# Autodesk Inventor assembly: 1103 Lift - Middle Tier
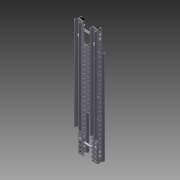
[picture p0: Inventor's stored thumbnail of the model, 180x180]
Saved by Autodesk Inventor 2012 (Build 160160000, 160)
## iProperties
Created: 2011-08-16
Part Number: 1103 Lift - Middle Tier
Document SubType Name: Assembly
Designer: Dakota.Bayer
Author: Dakota.Bayer
## Documents named in this file (11)
- C:\Users\Wade\Documents\1103 Robot - CAD Assembly\1103 Lift - Middle Tier.iam
- C:\Users\Wade\Documents\1103 Robot - CAD Assembly\Outside.ipt
- C:\Users\Wade\Documents\1103 Robot - CAD Assembly\1103 custom 5 x 30.ipt
- C:\Users\Wade\Documents\1103 Robot - CAD Assembly\Flat Bearing Block.ipt
- C:\Users\Wade\Documents\24C VEX CAD Files\Metal Other\Linear Slide Assembly-Parts\Linear Slide-Inner.ipt
- C:\Users\Wade\Documents\24C VEX CAD Files\Screws & Nuts\Screw 8-32 x 0.250''-Silver.ipt
- C:\Users\Wade\Documents\24C VEX CAD Files\Standoffs & Couplers\Standoff 0.50''.ipt
- C:\Users\Wade\Documents\1103 Robot - CAD Assembly\.5'' Screw & Nylock Nut.iam
- C:\Users\Wade\Documents\1103 Robot - CAD Assembly\.375'' Screw & Nylock Nut.iam
- C:\Users\Wade\Documents\24C VEX CAD Files\Screws & Nuts\Screw 8-32 x 0.500''-Silver.ipt
- C:\Users\Wade\Documents\24C VEX CAD Files\Standoffs & Couplers\Standoff 2.00''.ipt
## Components (35 placed, 10 different names)
1. Outside:1 — Mate:26, Flush:12, Mate:149, Mate:151
2. Outside:2 — Flush:25, Mate:153, Mate:154
3. Screw 8-32 x 0.250''-Silver:2
4. 1103 custom 5 x 30:1 — Mate:26, Flush:12, Mate:59, Mate:64, Mate:81, Mate:86, Flush:25, Mate:114, Mate:115, Mate:116, Mate:117, Mate:118, Mate:119, Mate:120, Mate:125, Mate:127, Mate:129, Mate:130, Mate:131, Mate:134, Mate:136, Mate:137, Mate:138, Mate:141, Mate:143, Mate:144, Mate:145, Mate:146, Mate:147, Mate:148, Mate:150, Mate:152, Mate:156, Mate:158, Mate:160, Mate:162
5. Standoff 0.50'':1
6. Standoff 0.50'':2
7. Standoff 0.50'':3
8. Standoff 0.50'':4
9. Linear Slide-Inner:1
10. Screw 8-32 x 0.250''-Silver:5
11. Screw 8-32 x 0.250''-Silver:6
12. Linear Slide-Inner:2
13. Screw 8-32 x 0.250''-Silver:7
14. Screw 8-32 x 0.250''-Silver:8
15. Flat Bearing Block:1 — Mate:59, Mate:118, Mate:119, Mate:120, Mate:121, Mate:161
16. Flat Bearing Block:2 — Mate:64, Mate:114, Mate:115, Mate:116, Mate:117, Mate:123, Mate:159, Mate:164
17. Flat Bearing Block:3 — Mate:81, Mate:136, Mate:137, Mate:138, Mate:139, Mate:157
18. Flat Bearing Block:4 — Mate:86, Mate:129, Mate:130, Mate:131, Mate:132, Mate:155, Mate:166
19. Screw 8-32 x 0.250''-Silver:9
20. Screw 8-32 x 0.250''-Silver:10
21. Screw 8-32 x 0.250''-Silver:11
22. .5'' Screw & Nylock Nut:1 [sub-assembly] — Mate:121, Mate:125
23. .5'' Screw & Nylock Nut:3 [sub-assembly] — Mate:123, Mate:127
24. .5'' Screw & Nylock Nut:5 [sub-assembly] — Mate:139, Mate:141
25. .5'' Screw & Nylock Nut:6 [sub-assembly] — Mate:132, Mate:134
26. Screw 8-32 x 0.500''-Silver:1 — Mate:155, Mate:156, Mate:165
27. .375'' Screw & Nylock Nut:1 [sub-assembly] — Mate:146, Mate:147, Mate:148
28. .375'' Screw & Nylock Nut:2 [sub-assembly] — Mate:143, Mate:144, Mate:145
29. .375'' Screw & Nylock Nut:3 [sub-assembly] — Mate:149, Mate:150, Mate:151
30. .375'' Screw & Nylock Nut:4 [sub-assembly] — Mate:152, Mate:153, Mate:154
31. Screw 8-32 x 0.500''-Silver:2 — Mate:157, Mate:158
32. Screw 8-32 x 0.500''-Silver:3 — Mate:161, Mate:162
33. Screw 8-32 x 0.500''-Silver:4 — Mate:159, Mate:160, Mate:163
34. Standoff 2.00'':1 — Mate:163, Mate:164
35. Standoff 2.00'':2 — Mate:165, Mate:166
## Relationships (91: Mate 76, Tangent 12, Flush 3)
- Mate:26: Outside:1 ↔ 1103 custom 5 x 30:1
- Flush:12: Outside:1 ↔ 1103 custom 5 x 30:1
- [Tangent] (0.2286 mm): Screw 8-32 x 0.250''-Silver:2 ↔ 1103 custom 5 x 30:1
- [Mate]: 1103 custom 5 x 30:1 ↔ Standoff 0.50'':1
- [Mate]: 1103 custom 5 x 30:1 ↔ Standoff 0.50'':2
- [Mate]: 1103 custom 5 x 30:1 ↔ Standoff 0.50'':3
- [Mate]: 1103 custom 5 x 30:1 ↔ Standoff 0.50'':4
- [Mate]: Screw 8-32 x 0.250''-Silver:2 ↔ Standoff 0.50'':4
- [Mate]: Standoff 0.50'':3 ↔ Linear Slide-Inner:1
- [Mate]: Linear Slide-Inner:1 ↔ Screw 8-32 x 0.250''-Silver:5
- [Tangent] (0.2286 mm): Linear Slide-Inner:1 ↔ Screw 8-32 x 0.250''-Silver:5
- [Mate]: Standoff 0.50'':1 ↔ Linear Slide-Inner:1
- [Mate]: Linear Slide-Inner:1 ↔ Screw 8-32 x 0.250''-Silver:6
- [Tangent] (0.2286 mm): Linear Slide-Inner:1 ↔ Screw 8-32 x 0.250''-Silver:6
- [Mate]: Standoff 0.50'':1 ↔ Screw 8-32 x 0.250''-Silver:6
- [Mate]: Standoff 0.50'':4 ↔ Linear Slide-Inner:2
- [Mate]: Standoff 0.50'':2 ↔ Linear Slide-Inner:2
- [Mate]: Linear Slide-Inner:2 ↔ Screw 8-32 x 0.250''-Silver:7
- [Tangent] (0.2286 mm): Linear Slide-Inner:2 ↔ Screw 8-32 x 0.250''-Silver:7
- [Mate]: Linear Slide-Inner:2 ↔ Screw 8-32 x 0.250''-Silver:8
- [Tangent] (0.2286 mm): Linear Slide-Inner:2 ↔ Screw 8-32 x 0.250''-Silver:8
- [Mate]: Standoff 0.50'':2 ↔ Screw 8-32 x 0.250''-Silver:7
- [Mate]: Standoff 0.50'':4 ↔ Screw 8-32 x 0.250''-Silver:8
- Mate:59: 1103 custom 5 x 30:1 ↔ Flat Bearing Block:1
- Mate:64: 1103 custom 5 x 30:1 ↔ Flat Bearing Block:2
- Mate:81: 1103 custom 5 x 30:1 ↔ Flat Bearing Block:3
- Mate:86: 1103 custom 5 x 30:1 ↔ Flat Bearing Block:4
- [Mate]: Standoff 0.50'':3 ↔ Screw 8-32 x 0.250''-Silver:5
- [Tangent] (0.2286 mm): Linear Slide-Inner:1 ↔ Screw 8-32 x 0.250''-Silver:6
- [Tangent] (0.2286 mm): Linear Slide-Inner:1 ↔ Screw 8-32 x 0.250''-Silver:5
- [Flush]: 1103 custom 5 x 30:1 ↔ Linear Slide-Inner:1
- [Mate]: Outside:1 ↔ Screw 8-32 x 0.250''-Silver:9
- [Tangent] (0.2286 mm): 1103 custom 5 x 30:1 ↔ Screw 8-32 x 0.250''-Silver:9
- [Tangent] (0.2286 mm): 1103 custom 5 x 30:1 ↔ Screw 8-32 x 0.250''-Silver:9
- [Mate]: Standoff 0.50'':1 ↔ Screw 8-32 x 0.250''-Silver:9
- [Mate]: Screw 8-32 x 0.250''-Silver:2 ↔ 1103 custom 5 x 30:1
- [Tangent] (0.2286 mm): Linear Slide-Inner:2 ↔ Screw 8-32 x 0.250''-Silver:8
- [Tangent] (0.2286 mm): Screw 8-32 x 0.250''-Silver:2 ↔ 1103 custom 5 x 30:1
- [Tangent] (0.2286 mm): Linear Slide-Inner:2 ↔ Screw 8-32 x 0.250''-Silver:7
- [Mate]: Outside:2 ↔ Screw 8-32 x 0.250''-Silver:10
- [Mate]: Standoff 0.50'':2 ↔ Screw 8-32 x 0.250''-Silver:10
- [Mate]: 1103 custom 5 x 30:1 ↔ Screw 8-32 x 0.250''-Silver:11
- [Mate]: Standoff 0.50'':3 ↔ Screw 8-32 x 0.250''-Silver:11
- [Mate] (2.3114 mm): 1103 custom 5 x 30:1 ↔ Standoff 0.50'':2
- [Mate] (1.1684 mm): 1103 custom 5 x 30:1 ↔ Screw 8-32 x 0.250''-Silver:10
- Flush:25: Outside:2 ↔ 1103 custom 5 x 30:1
- Mate:114 (2.3114 mm): 1103 custom 5 x 30:1 ↔ Flat Bearing Block:2
- Mate:115 (2.3114 mm): 1103 custom 5 x 30:1 ↔ Flat Bearing Block:2
- Mate:116 (2.3114 mm): 1103 custom 5 x 30:1 ↔ Flat Bearing Block:2
- Mate:117 (2.3114 mm): 1103 custom 5 x 30:1 ↔ Flat Bearing Block:2
- Mate:118 (2.3114 mm): 1103 custom 5 x 30:1 ↔ Flat Bearing Block:1
- Mate:119 (2.3114 mm): 1103 custom 5 x 30:1 ↔ Flat Bearing Block:1
- Mate:120 (2.3114 mm): 1103 custom 5 x 30:1 ↔ Flat Bearing Block:1
- Mate:121: Flat Bearing Block:1 ↔ .5'' Screw & Nylock Nut:1
- Mate:123: Flat Bearing Block:2 ↔ .5'' Screw & Nylock Nut:3
- Mate:125: 1103 custom 5 x 30:1 ↔ .5'' Screw & Nylock Nut:1
- Mate:127: 1103 custom 5 x 30:1 ↔ .5'' Screw & Nylock Nut:3
- Mate:129 (2.3114 mm): 1103 custom 5 x 30:1 ↔ Flat Bearing Block:4
- Mate:130 (2.3114 mm): 1103 custom 5 x 30:1 ↔ Flat Bearing Block:4
- Mate:131 (2.3114 mm): 1103 custom 5 x 30:1 ↔ Flat Bearing Block:4
- Mate:132: Flat Bearing Block:4 ↔ .5'' Screw & Nylock Nut:6
- Mate:134: 1103 custom 5 x 30:1 ↔ .5'' Screw & Nylock Nut:6
- Mate:136 (2.3114 mm): 1103 custom 5 x 30:1 ↔ Flat Bearing Block:3
- Mate:137 (2.3114 mm): 1103 custom 5 x 30:1 ↔ Flat Bearing Block:3
- Mate:138 (2.3114 mm): 1103 custom 5 x 30:1 ↔ Flat Bearing Block:3
- Mate:139: Flat Bearing Block:3 ↔ .5'' Screw & Nylock Nut:5
- Mate:141: 1103 custom 5 x 30:1 ↔ .5'' Screw & Nylock Nut:5
- Mate:143 (2.3114 mm): 1103 custom 5 x 30:1 ↔ .375'' Screw & Nylock Nut:2
- Mate:144 (2.3114 mm): 1103 custom 5 x 30:1 ↔ .375'' Screw & Nylock Nut:2
- Mate:145: 1103 custom 5 x 30:1 ↔ .375'' Screw & Nylock Nut:2
- Mate:146 (2.3114 mm): 1103 custom 5 x 30:1 ↔ .375'' Screw & Nylock Nut:1
- Mate:147 (2.3114 mm): 1103 custom 5 x 30:1 ↔ .375'' Screw & Nylock Nut:1
- Mate:148: 1103 custom 5 x 30:1 ↔ .375'' Screw & Nylock Nut:1
- Mate:149 (2.3114 mm): Outside:1 ↔ .375'' Screw & Nylock Nut:3
- Mate:150 (2.3114 mm): 1103 custom 5 x 30:1 ↔ .375'' Screw & Nylock Nut:3
- Mate:151: Outside:1 ↔ .375'' Screw & Nylock Nut:3
- Mate:152 (2.3114 mm): 1103 custom 5 x 30:1 ↔ .375'' Screw & Nylock Nut:4
- Mate:153 (2.3114 mm): Outside:2 ↔ .375'' Screw & Nylock Nut:4
- Mate:154: Outside:2 ↔ .375'' Screw & Nylock Nut:4
- Mate:155: Flat Bearing Block:4 ↔ Screw 8-32 x 0.500''-Silver:1
- Mate:156: 1103 custom 5 x 30:1 ↔ Screw 8-32 x 0.500''-Silver:1
- Mate:157: Flat Bearing Block:3 ↔ Screw 8-32 x 0.500''-Silver:2
- Mate:158: 1103 custom 5 x 30:1 ↔ Screw 8-32 x 0.500''-Silver:2
- Mate:159: Flat Bearing Block:2 ↔ Screw 8-32 x 0.500''-Silver:4
- Mate:160: 1103 custom 5 x 30:1 ↔ Screw 8-32 x 0.500''-Silver:4
- Mate:161: Flat Bearing Block:1 ↔ Screw 8-32 x 0.500''-Silver:3
- Mate:162: 1103 custom 5 x 30:1 ↔ Screw 8-32 x 0.500''-Silver:3
- Mate:163: Screw 8-32 x 0.500''-Silver:4 ↔ Standoff 2.00'':1
- Mate:164: Flat Bearing Block:2 ↔ Standoff 2.00'':1
- Mate:165: Screw 8-32 x 0.500''-Silver:1 ↔ Standoff 2.00'':2
- Mate:166: Flat Bearing Block:4 ↔ Standoff 2.00'':2
